# Autodesk Inventor assembly: assembly
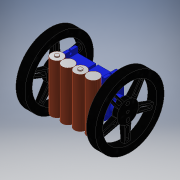
[picture p0: Inventor's stored thumbnail of the model, 180x180]
Saved by Autodesk Inventor 2016 (Build 200138000, 138)
## iProperties
Created: 2016-01-12
Part Number: assembly
Document SubType Name: Assembly
Designer: jferner
Author: jferner
## Documents named in this file (4)
- C:\dev\minirobot\mechanical\assembly.iam
- C:\dev\minirobot\mechanical\micro-servo.ipt
- C:\dev\minirobot\mechanical\wheel.ipt
- C:\dev\minirobot\mechanical\battery-aaa.ipt
## Components (8 placed, 3 different names)
1. micro-servo:1 — Mate:1, Flush:1, Flush:2, Mate:2, Insert:2, Mate:3
2. micro-servo:2 — Mate:1, Flush:1, Flush:2, Insert:1, Flush:6
3. wheel:1 — Insert:2
4. wheel:2 — Insert:1
5. battery-aaa:1 — Tangent:2, Tangent:3, Flush:4, Flush:5
6. battery-aaa:2 — Tangent:1, Tangent:2, Flush:3, Flush:4
7. battery-aaa:3 — Tangent:1, Flush:3, Flush:6
8. battery-aaa:4 — Tangent:3, Flush:5
## Relationships (14: Flush 6, Mate 3, Tangent 3, Insert 2)
- Mate:1 (2 mm): micro-servo:1 ↔ micro-servo:2
- Flush:1: micro-servo:1 ↔ micro-servo:2
- Flush:2: micro-servo:1 ↔ micro-servo:2
- Mate:2: micro-servo:1
- Insert:1: micro-servo:2 ↔ wheel:2
- Insert:2: micro-servo:1 ↔ wheel:1
- Mate:3: micro-servo:1
- Tangent:1: battery-aaa:2 ↔ battery-aaa:3
- Tangent:2: battery-aaa:1 ↔ battery-aaa:2
- Tangent:3: battery-aaa:1 ↔ battery-aaa:4
- Flush:3: battery-aaa:2 ↔ battery-aaa:3
- Flush:4: battery-aaa:1 ↔ battery-aaa:2
- Flush:5: battery-aaa:1 ↔ battery-aaa:4
- Flush:6 (11 mm): micro-servo:2 ↔ battery-aaa:3
